# Autodesk Inventor assembly: jokez
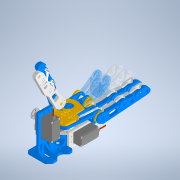
[picture p0: Inventor's stored thumbnail of the model, 180x180]
Saved by Autodesk Inventor 2020.3 (Build 243373000, 373)
## iProperties
Created: 2019-09-17
Part Number: jokez
Document SubType Name: Assembly
Designer: Horváth Patrik
Author: Horváth Patrik
## Documents named in this file (12)
- E:\Dokumentumok\Simonyi\INDACT\Robotarm - kézfej fileok\kéz12.0\jokez.iam
- E:\Dokumentumok\Simonyi\INDACT\Robotarm - kézfej fileok\kéz12.0\motor_sima.iam
- E:\Dokumentumok\Simonyi\INDACT\Robotarm - kézfej fileok\kéz12.0\ujj_alapmodell.iam
- E:\Dokumentumok\Simonyi\INDACT\Robotarm - kézfej fileok\kéz12.0\Part2.ipt
- E:\Dokumentumok\Simonyi\INDACT\Robotarm - kézfej fileok\kéz12.0\Part3.ipt
- C:\Users\Horváth Patrik\Documents\Inventor\Content Center Files\R2020\en-US\ISO 4762(2)\ISO 4762 - M2 x 16ISO.ipt
- C:\Users\Horváth Patrik\Documents\Inventor\Content Center Files\R2020\en-US\ISO 4032(2)\ISO 4032 - M2 - ISO.ipt
- C:\Users\Horváth Patrik\Documents\Inventor\Content Center Files\R2020\en-US\ISO 4762(2)\ISO 4762 - M4 x 10ISO.ipt
- E:\Dokumentumok\Simonyi\INDACT\Robotarm - kézfej fileok\kéz12.0\kezfej_1.iam
- E:\Dokumentumok\Simonyi\INDACT\Robotarm - kézfej fileok\kéz12.0\Part6.ipt
- E:\Dokumentumok\Simonyi\INDACT\Robotarm - kézfej fileok\kéz12.0\Solid4_1.ipt
- C:\Users\Horváth Patrik\Documents\Inventor\Content Center Files\R2020\en-US\ISO 4762(2)\ISO 4762 - M2 x 20ISO.ipt
## Components (19 placed, 11 different names)
1. kezfej_1:2 [sub-assembly] — Mate:48, Mate:49, Mate:50, Mate:51, Mate:52, Mate:53, Mate:54, Mate:55, Mate:56, Mate:57, Mate:58, Mate:59, Mate:60, Mate:61, Mate:62, Mate:63, Mate:64, Mate:65, Mate:66, Angle:1, Mate:70, Mate:71, Mate:72, Mate:73, Mate:74, Mate:75
2. motor_sima:1 [sub-assembly] — Mate:48, Mate:49, Mate:50, Mate:69
3. motor_sima:2 [sub-assembly] — Mate:31, Mate:46, Mate:47, Mate:51, Mate:52, Mate:53
4. motor_sima:3 [sub-assembly] — Mate:25, Mate:54, Mate:55, Mate:56
5. ujj_alapmodell:1 [sub-assembly] — Flush:1, Mate:61, Mate:62, Mate:70
6. ujj_alapmodell:2 [sub-assembly] — Flush:1, Mate:59, Mate:60, Angle:1, Mate:67, Mate:68, Mate:71
7. ujj_alapmodell:3 [sub-assembly] — Flush:2, Mate:39, Mate:40, Mate:63, Mate:65
8. ujj_alapmodell:4 [sub-assembly] — Mate:29, Mate:30, Flush:2, Mate:37, Mate:38, Mate:41, Mate:64, Mate:66
9. ujj_alapmodell:5 [sub-assembly] — Mate:23, Mate:24, Mate:57, Mate:58, Mate:74
10. Part2:1 — Mate:29, Mate:30, Mate:31, Mate:76
11. Part3:1 — Mate:23, Mate:24, Mate:25
12. ISO 4762 M2 x 16:1 — Mate:37, Mate:38, Mate:42
13. ISO 4762 M2 x 16:2 — Mate:39, Mate:40
14. ISO 4032 M2:1 — Mate:41, Mate:42
15. ISO 4762 M4 x 10:1 — Mate:46, Mate:47
16. ISO 4032 M2:2
17. Part6:1 — Mate:67, Mate:68, Mate:69
18. Solid4_1:1 — Mate:72, Mate:73
19. ISO 4762 M2 x 20:1 — Mate:75, Mate:76
## Relationships (46: Mate 43, Flush 2, Angle 1)
- Mate:23: ujj_alapmodell:5 ↔ Part3:1
- Mate:24: ujj_alapmodell:5 ↔ Part3:1
- Mate:25: motor_sima:3 ↔ Part3:1
- Flush:1: ujj_alapmodell:1 ↔ ujj_alapmodell:2
- Mate:29: ujj_alapmodell:4 ↔ Part2:1
- Mate:30: ujj_alapmodell:4 ↔ Part2:1
- Mate:31: motor_sima:2 ↔ Part2:1
- Flush:2: ujj_alapmodell:3 ↔ ujj_alapmodell:4
- Mate:37: ujj_alapmodell:4 ↔ ISO 4762 M2 x 16:1
- Mate:38: ujj_alapmodell:4 ↔ ISO 4762 M2 x 16:1
- Mate:39: ujj_alapmodell:3 ↔ ISO 4762 M2 x 16:2
- Mate:40: ujj_alapmodell:3 ↔ ISO 4762 M2 x 16:2
- Mate:41: ujj_alapmodell:4 ↔ ISO 4032 M2:1
- Mate:42: ISO 4762 M2 x 16:1 ↔ ISO 4032 M2:1
- Mate:46: motor_sima:2 ↔ ISO 4762 M4 x 10:1
- Mate:47: motor_sima:2 ↔ ISO 4762 M4 x 10:1
- Mate:48: kezfej_1:2 ↔ motor_sima:1
- Mate:49: kezfej_1:2 ↔ motor_sima:1
- Mate:50: kezfej_1:2 ↔ motor_sima:1
- Mate:51: kezfej_1:2 ↔ motor_sima:2
- Mate:52: kezfej_1:2 ↔ motor_sima:2
- Mate:53: kezfej_1:2 ↔ motor_sima:2
- Mate:54: kezfej_1:2 ↔ motor_sima:3
- Mate:55: kezfej_1:2 ↔ motor_sima:3
- Mate:56: kezfej_1:2 ↔ motor_sima:3
- Mate:57: kezfej_1:2 ↔ ujj_alapmodell:5
- Mate:58: kezfej_1:2 ↔ ujj_alapmodell:5
- Mate:59: kezfej_1:2 ↔ ujj_alapmodell:2
- Mate:60: kezfej_1:2 ↔ ujj_alapmodell:2
- Mate:61: kezfej_1:2 ↔ ujj_alapmodell:1
- Mate:62: kezfej_1:2 ↔ ujj_alapmodell:1
- Mate:63: kezfej_1:2 ↔ ujj_alapmodell:3
- Mate:64: kezfej_1:2 ↔ ujj_alapmodell:4
- Mate:65: kezfej_1:2 ↔ ujj_alapmodell:3
- Mate:66: kezfej_1:2 ↔ ujj_alapmodell:4
- Angle:1 (0 deg): kezfej_1:2 ↔ ujj_alapmodell:2
- Mate:67: ujj_alapmodell:2 ↔ Part6:1
- Mate:68: ujj_alapmodell:2 ↔ Part6:1
- Mate:69: motor_sima:1 ↔ Part6:1
- Mate:70: kezfej_1:2 ↔ ujj_alapmodell:1
- Mate:71: kezfej_1:2 ↔ ujj_alapmodell:2
- Mate:72: kezfej_1:2 ↔ Solid4_1:1
- Mate:73: kezfej_1:2 ↔ Solid4_1:1
- Mate:74: kezfej_1:2 ↔ ujj_alapmodell:5
- Mate:75: kezfej_1:2 ↔ ISO 4762 M2 x 20:1
- Mate:76: Part2:1 ↔ ISO 4762 M2 x 20:1
